# Autodesk Inventor assembly: Base
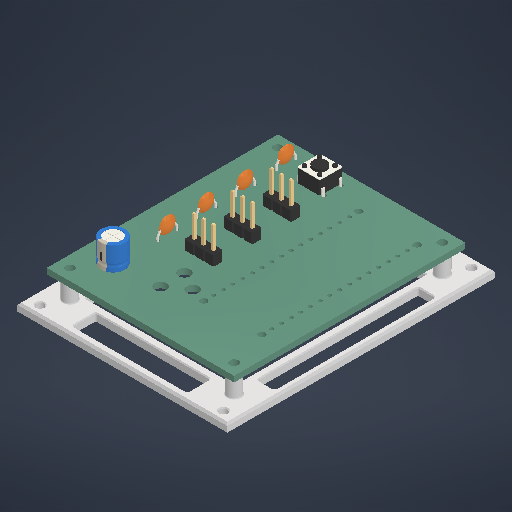
[picture p0: Inventor's stored thumbnail of the model, 512x512]
Saved by Autodesk Inventor 2026 (Build 300175000, 175)
## iProperties
Created: 2026-02-15
Part Number: Base
Document SubType Name: Assembly
Designer: Jakob Dorninger
Author: Jakob Dorninger
## Documents named in this file (3)
- C:\05_Projekte\Articulated-Robot\CAD\Base.iam
- C:\05_Projekte\Articulated-Robot\CAD\PCB.ipt
- C:\05_Projekte\Articulated-Robot\CAD\PCB-Base.ipt
## Components (2 placed, 2 different names)
1. PCB:1 — Passend:1, Passend:2, Passend:3
2. PCB-Base:1 — Passend:1, Passend:2, Passend:3
## Relationships (3: Mate 3)
- Passend:1 [Mate]: PCB:1 ↔ PCB-Base:1
- Passend:2 [Mate]: PCB:1 ↔ PCB-Base:1
- Passend:3 [Mate]: PCB:1 ↔ PCB-Base:1
